# Autodesk Inventor assembly: アーム先端
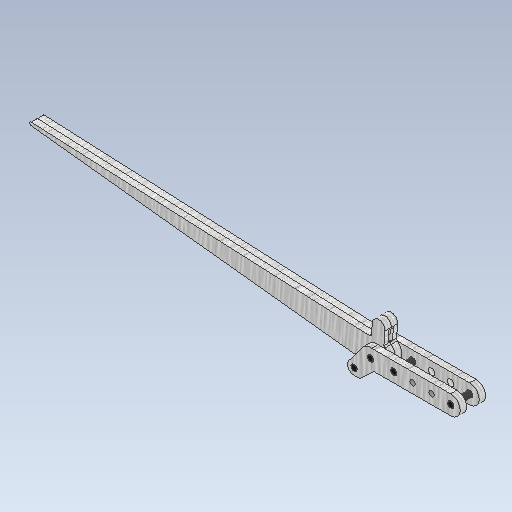
[picture p0: Inventor's stored thumbnail of the model, 512x512]
Saved by Autodesk Inventor 2020.2 (Build 242310000, 310)
## iProperties
Created: 2020-03-28
Part Number: アーム先端
Document SubType Name: Assembly
Designer: aoyam
Mass: 29.5511 g
Surface Area: 117.169 cm^2
Volume: 9.75011 cm^3
Density: 3.03085 g/cm^3
Author: aoyam
## Documents named in this file (8)
- C:\Users\aoyam\Desktop\SRDC_local\Inventor\二年機\Geminiβ\腕\アーム先端.iam
- C:\Users\aoyam\Desktop\SRDC_local\Inventor\二年機\Geminiβ\腕\中間節アーム先端締結パーツipt.ipt
- C:\Users\aoyam\Desktop\SRDC_local\Inventor\二年機\Geminiβ\腕\アーム先端.ipt
- C:\Users\aoyam\Desktop\SRDC_local\Inventor\二年機\Geminiβ\汎用部品\スペーサー中空M3L6アルミ.ipt
- C:\Users\aoyam\Desktop\SRDC_local\Inventor\二年機\Geminiβ\汎用部品\オイレスd6D8L6.ipt
- C:\Users\aoyam\Desktop\SRDC_local\Inventor\二年機\Geminiβ\腕\中間節アーム先端締結パーツ外.ipt
- C:\Users\aoyam\Desktop\SRDC_local\Inventor\二年機\Geminiβ\汎用部品\ネジボタンM3L12.ipt
- C:\Users\aoyam\Desktop\SRDC_local\Inventor\二年機\Geminiβ\腕\MIR達\MIRアーム先端.ipt
## Components (11 placed, 7 different names)
1. 中間節アーム先端締結パーツipt:2 — 挿入:5, 挿入:8, 挿入:11, 挿入:12, 挿入:13, 挿入:14
2. アーム先端:2 — 挿入:15, 挿入:17, フラッシュ:1
3. スペーサー中空M3L6アルミ:1 — 挿入:8, 挿入:9
4. スペーサー中空M3L6アルミ:2 — 挿入:5, 挿入:10, 挿入:16
5. オイレスd6D8L6:1 — 挿入:15, 挿入:16
6. 中間節アーム先端締結パーツ外:1 — 挿入:9, 挿入:10
7. ネジボタンM3L12:1 — 挿入:11
8. ネジボタンM3L12:2 — 挿入:13
9. ネジボタンM3L12:3 — 挿入:12
10. ネジボタンM3L12:4 — 挿入:14
11. MIRアーム先端:1 — 挿入:17, フラッシュ:1
## Relationships (12: Insert 11, Flush 1)
- 挿入:5 [Insert]: 中間節アーム先端締結パーツipt:2 ↔ スペーサー中空M3L6アルミ:2
- 挿入:8 [Insert]: 中間節アーム先端締結パーツipt:2 ↔ スペーサー中空M3L6アルミ:1
- 挿入:9 [Insert]: スペーサー中空M3L6アルミ:1 ↔ 中間節アーム先端締結パーツ外:1
- 挿入:10 [Insert]: スペーサー中空M3L6アルミ:2 ↔ 中間節アーム先端締結パーツ外:1
- 挿入:11 [Insert]: 中間節アーム先端締結パーツipt:2 ↔ ネジボタンM3L12:1
- 挿入:12 [Insert]: 中間節アーム先端締結パーツipt:2 ↔ ネジボタンM3L12:3
- 挿入:13 [Insert]: 中間節アーム先端締結パーツipt:2 ↔ ネジボタンM3L12:2
- 挿入:14 [Insert]: 中間節アーム先端締結パーツipt:2 ↔ ネジボタンM3L12:4
- 挿入:15 [Insert]: アーム先端:2 ↔ オイレスd6D8L6:1
- 挿入:16 [Insert]: スペーサー中空M3L6アルミ:2 ↔ オイレスd6D8L6:1
- 挿入:17 [Insert]: アーム先端:2 ↔ MIRアーム先端:1
- フラッシュ:1 [Flush]: アーム先端:2 ↔ MIRアーム先端:1
